# Autodesk Inventor assembly: m4 bearing assembly 30mm
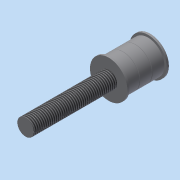
[picture p0: Inventor's stored thumbnail of the model, 180x180]
Saved by Autodesk Inventor 2015 (Build 190159000, 159)
## iProperties
Created: 2016-09-08
Part Number: m4 bearing assembly 30mm
Document SubType Name: Assembly
Designer: Dustin
Author: Dustin
## Documents named in this file (4)
- E:\Documents\3D Printer\LetzteBot3DPrinter\Inventor Files\IAM Files\m4 bearing assembly 30mm.iam
- E:\Documents\3D Printer\Parts\New Printer\8x4x3 bearing.ipt
- E:\Documents\3D Printer\Parts\New Printer\m4x30.ipt
- E:\Documents\3D Printer\Parts\New Printer\washer.ipt
## Components (6 placed, 3 different names)
1. 8x4x3 bearing:1 — Mate:3, Insert:3, Insert:5
2. 8x4x3 bearing:2 — Mate:2, Mate:3, Insert:2, Insert:3
3. 8x4x3 bearing:3 — Mate:2, Insert:1, Insert:2
4. m4x30:1 — Insert:1, Insert:4
5. washer:1 — Insert:4
6. washer:2 — Insert:5
## Relationships (7: Insert 5, Mate 2)
- Mate:2: 8x4x3 bearing:2 ↔ 8x4x3 bearing:3
- Mate:3: 8x4x3 bearing:1 ↔ 8x4x3 bearing:2
- Insert:1 (0.5 mm): 8x4x3 bearing:3 ↔ m4x30:1
- Insert:2: 8x4x3 bearing:2 ↔ 8x4x3 bearing:3
- Insert:3: 8x4x3 bearing:1 ↔ 8x4x3 bearing:2
- Insert:4: m4x30:1 ↔ washer:1
- Insert:5: 8x4x3 bearing:1 ↔ washer:2
